# Autodesk Inventor assembly: 000 Ensamblaje hw_DAA - PCB Power
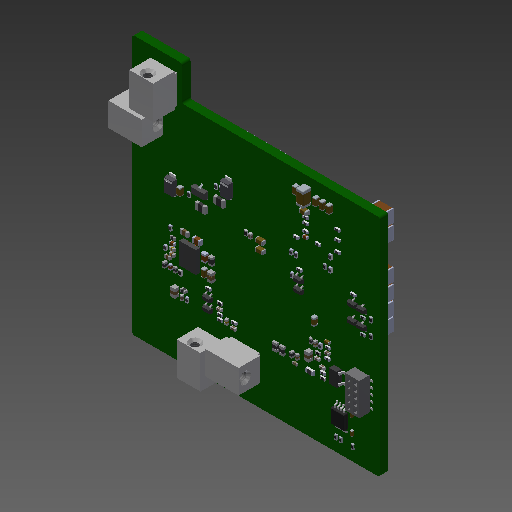
[picture p0: Inventor's stored thumbnail of the model, 512x512]
Saved by Autodesk Inventor 2018 (Build 220112000, 112)
## iProperties
Created: 2024-03-13
Part Number: 000 Ensamblaje hw_DAA - PCB Power
Document SubType Name: Assembly
Designer: cda1
Author: cda1
## Documents named in this file (82)
- C:\Users\cda1\Git\DAA\items\hw_DAA\variants\BASIC\3d\000 Ensamblaje hw_DAA - PCB Power.iam
- C:\Users\cda1\Git\DAA\items\hw_DAA\3d\hw_DAA - PCB Power.ipt
- C:\Users\cda1\Git\DAA\items\_accessories\Componentes PCB\Capacitadores\3d_TDK\3d\CGA9N3X7S2A106K230KB\CGA9N3X7S2A106K230KB.iam
- C:\Users\cda1\Git\DAA\items\_accessories\Componentes PCB\Bobinas\3d_COILCRAFT\3d\XAL7030-472MEC\XAL7030-472MEC.iam
- C:\Users\cda1\Git\DAA\items\_accessories\Componentes PCB\PMIC\TPS65930400RWERQ1\TPS65930400RWERQ1.iam
- C:\Users\cda1\Git\DAA\items\_accessories\Componentes PCB\Mosfet\3d_Vishay\3d\SQJ402EP-T1_GE3.ipt
- C:\Users\cda1\Git\DAA\items\_accessories\Componentes PCB\Mosfet\3d_Vishay\3d\SQJ465EP-T1_GE3\SQJ465EP-T1_GE3.ipt
- C:\Users\cda1\Git\DAA\items\_accessories\Componentes PCB\Inductor\3d_Coilcraft\3d\XAL5030-222MEC\XAL5030-222MEC.ipt
- C:\Users\cda1\Git\DAA\items\_accessories\Componentes PCB\Inductor\3d_Coilcraft\3d\XFL4020-152MEC\XFL4020-152MEC.iam
- C:\Users\cda1\Git\DAA\items\_accessories\Componentes PCB\Inductor\3d_Coilcraft\3d\XEL4020-101MEC\XEL4020-101MEC.iam
- C:\Users\cda1\Git\DAA\items\_accessories\Componentes PCB\Inductor\3d_TDK\3d\XAL4020-601MEC\XAL4020-601MEC.ipt
- C:\Users\cda1\Git\DAA\items\_accessories\Componentes PCB\Capacitadores\3d_Murata Electronics\3d\GCM32EC71A476KE02K\GCM32EC71A476KE02K.ipt
- C:\Users\cda1\Git\DAA\items\_accessories\Componentes PCB\Inductor\3d_TDK\3d\TFM322512ALMAR22MTAA\TFM322512ALMAR22MTAA.iam
- C:\Users\cda1\Git\DAA\items\_accessories\Componentes PCB\Inductor\3d_TDK\3d\TFM322512ALMAR47MTAA\TFM322512ALMAR47MTAA.iam
- C:\Users\cda1\Git\DAA\items\_accessories\Componentes PCB\DC-DC\3d_Texas Instruments\3d\TPS54116QRTWTQ1\TPS54116QRTWTQ1.iam
- C:\Users\cda1\Git\DAA\items\_accessories\Componentes PCB\Conversores\Buck converter\3d_Texas_instruments\TPS62873QWRXSRQ1.iam
- C:\Users\cda1\Git\DAA\items\_accessories\Componentes PCB\Analog Switch\3d_Texas_Instruments\TS5A23157TDGSRQ1\TS5A23157TDGSRQ1.iam
- C:\Users\cda1\Git\DAA\items\_accessories\Componentes PCB\Capacitadores\3d_Taiyo Yuden\3d\EMK212BBJ106KGHT.ipt
- C:\Users\cda1\Git\DAA\items\_accessories\Componentes PCB\Capacitadores\3d_Murata Electronics\3d\GRT32ER60J107ME13L.ipt
- C:\Users\cda1\Git\DAA\items\_accessories\Componentes PCB\Condensadores\3d_TDK\3d\CGA6P3X7S1H685M250AB\CGA6P3X7S1H685M250AB.iam
- C:\Users\cda1\Git\DAA\items\_accessories\Componentes PCB\Capacitadores\3d_Murata Electronics\3d\GRM31CC72A475ME11L.ipt
- C:\Users\cda1\Git\DAA\items\_accessories\Componentes PCB\Reguladores\3d_Texas Instruments\3d\TPS57112CQRTERQ1\TPS57112CQRTERQ1.iam
- C:\Users\cda1\Git\DAA\items\_accessories\Componentes PCB\Reguladores\3d_Texas Instruments\3d\TPS74525PQWDRBRQ1\TPS74525PQWDRBRQ1.iam
- C:\Users\cda1\Git\DAA\items\_accessories\Componentes PCB\Cristales\3d_ECS\3d\ECS-.327-12.5-34QCS-TR\ECS-.327-12.5-34QCS-TR.ipt
- C:\Users\cda1\Git\DAA\items\_accessories\Componentes PCB\Diodos\3d_Semtech\3d\RCLAMP3324PQTCT\RCLAMP3324PQTCT.ipt
- C:\Users\cda1\Git\DAA\items\_accessories\Componentes PCB\Resistencias\3d_Vishay\3d\CRCW12061R00FKEAHP\CRCW12061R00FKEAHP.iam
- C:\Users\cda1\Git\DAA\items\_accessories\Componentes PCB\Resistencias\3d_Vishay\3d\CMB02070X1000GB200\CMB02070X1000GB200.ipt
- C:\Users\cda1\Git\DAA\items\_accessories\Componentes PCB\Capacitadores\3d_TDK\3d\CGA3E1X7S1C225K080AC\CGA3E1X7S1C225K080AC.iam
- C:\Users\cda1\Git\DAA\items\_accessories\Componentes PCB\Capacitadores\3d_Murata Electronics\3d\GCM1555C1H120JA16J\GCM1555C1H120JA16J.iam
- C:\Users\cda1\Git\DAA\items\_accessories\Componentes PCB\Capacitadores\3d_TDK\3d\CGA2B3X7R1H104K050BD.ipt
- C:\Users\cda1\Git\DAA\items\_accessories\Componentes PCB\Capacitadores\3d_Murata Electronics\3d\GRT188C81A106ME13D.ipt
- C:\Users\cda1\Git\DAA\items\_accessories\Componentes PCB\Capacitadores\3d_Taiyo Yuden\3d\HMJ107BB7104KAHT.ipt
- C:\Users\cda1\Git\DAA\items\_accessories\Componentes PCB\Capacitadores\3d_Genérico\3d\CAPC-0402-T0.55-BN.ipt
- C:\Users\cda1\Git\DAA\items\_accessories\Componentes PCB\Capacitadores\3d_Murata Electronics\3d\GCM1555C1H121JA16D\GCM1555C1H121JA16D.ipt
- C:\Users\cda1\Git\DAA\items\_accessories\Componentes PCB\Resistencias\3d_Panasonic\3d\ERJ-2GE0R00X.ipt
- C:\Users\cda1\Git\DAA\items\_accessories\Componentes PCB\Resistencias\3d_Panasonic\3d\ERJ-2RKF2002X\ERJ-2RKF2002X.iam
- C:\Users\cda1\Git\DAA\items\_accessories\Componentes PCB\Resistencias\3d_Vishay\3d\CRCW04028K66FKTD\CRCW04028K66FKTD.ipt
- C:\Users\cda1\Git\DAA\items\_accessories\Componentes PCB\Resistencias\3d_Panasonic\3d\ERJ-2RKF1543X\ERJ-2RKF1543X.iam
- C:\Users\cda1\Git\DAA\items\_accessories\Componentes PCB\Resistencias\3d_Genérico\RESC-0402.ipt
- C:\Users\cda1\Git\DAA\items\_accessories\Componentes PCB\Resistencias\3d_Panasonic\3d\ERJ-2RKF1002X.ipt
- C:\Users\cda1\Git\DAA\items\_accessories\Componentes PCB\Conectores\3d_Samtec\3d\CLP-105-02-F-D-BE\CLP-105-02-F-D-BE.iam
- C:\Users\cda1\Git\DAA\items\_accessories\Componentes PCB\Capacitadores\3d_Murata Electronics\3d\GRT31CC81C226KE01L.ipt
- C:\Users\cda1\Git\DAA\items\_accessories\Componentes PCB\Elementos mecanicos soldables\3d_Wurth Electronics\3d\SMD\WP-SMRA Redcube (M2) 7466302.ipt
- C:\Users\cda1\Git\DAA\items\_accessories\Componentes PCB\Elementos mecanicos soldables\3d_Wurth Electronics\3d\SMD\WP-SMRA Redcube (M2) 746630200.ipt
- C:\Users\cda1\Git\DAA\items\_accessories\Componentes PCB\DC-DC\3d_Texas Instruments\3d\LM5146QRGYRQ1\LM5146QRGYRQ1.iam
- C:\Users\cda1\Git\DAA\items\_accessories\Componentes PCB\I2C\3d_Texas_Instruments\TCA9517DGKRQ1\TCA9517DGKRQ1.iam
- C:\Users\cda1\Git\DAA\items\_accessories\Componentes PCB\Diodos\3d_Diodes Incorporated\3d\DMN2710UTQ-7\DMN2710UTQ-7.ipt
- C:\Users\cda1\Git\DAA\items\_accessories\Componentes PCB\Mosfet\3d_Infineon\3d\BSS123NH6327XTSA1\BSS123NH6327XTSA1.iam
- C:\Users\cda1\Git\DAA\items\_accessories\Componentes PCB\Diodos\3d_Vishay\3d\BZD27C10P-HE3-08.ipt
- C:\Users\cda1\Git\DAA\items\_accessories\Componentes PCB\Capacitadores\3d_Kemet\3d\C0603C105K4RACAUTO.ipt
- C:\Users\cda1\Git\DAA\items\_accessories\Componentes PCB\Capacitadores\3d_TDK\3d\CGA2B1X7S1C474K050BC.ipt
- C:\Users\cda1\Git\DAA\items\_accessories\Componentes PCB\Capacitadores\3d_Murata Electronics\3d\GCM155R71C563KA55J\GCM155R71C563KA55J.ipt
- C:\Users\cda1\Git\DAA\items\_accessories\Componentes PCB\Capacitadores\3d_Kemet\3d\C0402C822K4RACAUTO\C0402C822K4RACAUTO.ipt
- C:\Users\cda1\Git\DAA\items\_accessories\Componentes PCB\Capacitadores\3d_Murata Electronics\3d\GCG155R71H821KA01D\GCG155R71H821KA01D.ipt
- C:\Users\cda1\Git\DAA\items\_accessories\Componentes PCB\Capacitadores\3d_Murata Electronics\3d\GCM155R71H391KA37D\GCM155R71H391KA37D.ipt
- C:\Users\cda1\Git\DAA\items\_accessories\Componentes PCB\Capacitadores\3d_Kyocera\3d\06031A6R8J4T4A\06031A6R8J4T4A.ipt
- C:\Users\cda1\Git\DAA\items\_accessories\Componentes PCB\Capacitadores\3d_Kemet\3d\C0603X272J5GAC7867\C0603X272J5GAC7867.ipt
- C:\Users\cda1\Git\DAA\items\_accessories\Componentes PCB\Capacitadores\3d_TDK\3d\CGA2B1X7R1V224K050BC\CGA2B1X7R1V224K050BC.iam
- C:\Users\cda1\Git\DAA\items\_accessories\Componentes PCB\Capacitadores\3d_Murata Electronics\3d\GRT155R71H331KE01D\GRT155R71H331KE01D.ipt
- C:\Users\cda1\Git\DAA\items\_accessories\Componentes PCB\Capacitadores\3d_AVX\3d\04025A220C4T2A.ipt
- C:\Users\cda1\Git\DAA\items\_accessories\Componentes PCB\Capacitadores\3d_Murata Electronics\3d\GCM155R71H332KA37J\GCM155R71H332KA37J.ipt
- C:\Users\cda1\Git\DAA\items\_accessories\Componentes PCB\Capacitadores\3d_Murata Electronics\3d\GCQ1555C1H100FB01D\GCQ1555C1H100FB01D.ipt
- C:\Users\cda1\Git\DAA\items\_accessories\Componentes PCB\Condensadores\3d-Murata\3d\GCM155R72A472MA37D\GCM155R72A472MA37D.ipt
- C:\Users\cda1\Git\DAA\items\_accessories\Componentes PCB\Resistencias\3d_Yageo\3d\AC0805FR-0749K9L\AC0805FR-0749K9L.ipt
- C:\Users\cda1\Git\DAA\items\_accessories\Componentes PCB\Resistencias\3d_Panasonic\3d\ERJ-2RKF1003X.ipt
- C:\Users\cda1\Git\DAA\items\_accessories\Componentes PCB\Resistencias\3d_Panasonic\3d\ERJ-U02F4701X\ERJ-U02F4701X.iam
- C:\Users\cda1\Git\DAA\items\_accessories\Componentes PCB\Resistencias\3d_Vishay\3d\CRCW040233K0FKED\CRCW040233K0FKED.ipt
- C:\Users\cda1\Git\DAA\items\_accessories\Componentes PCB\Diodos\3d_Vishay\3d\GSOT05C-HE3-08.ipt
- C:\Users\cda1\Git\DAA\items\_accessories\Componentes PCB\Resistencias\3d_Vishay\3d\CRCW060315K0FKEA.ipt
- C:\Users\cda1\Git\DAA\items\_accessories\Componentes PCB\Resistencias\3d_Panasonic\3d\ERJ-2RKF9090X\ERJ-2RKF9090X.ipt
- C:\Users\cda1\Git\DAA\items\_accessories\Componentes PCB\Resistencias\3d_Vishay\3d\CRCW06036K19FKEA\CRCW06036K19FKEA.ipt
- C:\Users\cda1\Git\DAA\items\_accessories\Componentes PCB\Resistencias\3d_TE Connectivity\3d\CRGP0402F47K.ipt
- C:\Users\cda1\Git\DAA\items\_accessories\Componentes PCB\Resistencias\3d_Vishay\3d\CRCW0402110KFKTD\CRCW0402110KFKTD.ipt
- C:\Users\cda1\Git\DAA\items\_accessories\Componentes PCB\Resistencias\3d_Yageo\3d\AC0402FR-0797K6L.ipt
- C:\Users\cda1\Git\DAA\items\_accessories\Componentes PCB\Resistencias\3d_Vishay\3d\CRCW040278K7FKTD\CRCW040278K7FKTD.ipt
- C:\Users\cda1\Git\DAA\items\_accessories\Componentes PCB\Resistencias\3d_Vishay\3d\CRCW04023K40FKED\CRCW04023K40FKED.ipt
- C:\Users\cda1\Git\DAA\items\_accessories\Componentes PCB\Resistencias\3d_Vishay\3d\CRCW0402133RFKED\CRCW0402133RFKED.ipt
- C:\Users\cda1\Git\DAA\items\_accessories\Componentes PCB\Resistencias\3d_KOA\3d\RK73H1ETTP1802F\RK73H1ETTP1802F.ipt
- C:\Users\cda1\Git\DAA\items\_accessories\Componentes PCB\Resistencias\3d_Panasonic\3d\ERJ-2RKF1501X.ipt
- C:\Users\cda1\Git\DAA\items\_accessories\Componentes PCB\Resistencias\3d_Vishay\3d\CRCW040239K2FKED\CRCW040239K2FKED.ipt
- C:\Users\cda1\Git\DAA\items\_accessories\Componentes PCB\Resistencias\3d_Vishay\3d\CRCW06032R10FKEA\CRCW06032R10FKEA.ipt
- C:\Users\cda1\Git\DAA\items\_accessories\Componentes PCB\Resistencias\3d_Vishay\3d\CRCW0603931RFKEA\CRCW0603931RFKEA.ipt
## Components (216 placed, 81 different names)
1. hw_DAA - PCB Power:1 — Coincidencia:51, Coincidencia:52, Coincidencia:53, Coincidencia:54, Coincidencia:55, Coincidencia:56, Coincidencia:57, Coincidencia:58, Coincidencia:59, Coincidencia:60, Coincidencia:61, Coincidencia:62, Coincidencia:63, Coincidencia:64, Coincidencia:65, Coincidencia:66, Coincidencia:67, Coincidencia:68, Coincidencia:69, Coincidencia:70, Coincidencia:71, Coincidencia:72, Coincidencia:73, Coincidencia:74, Coincidencia:75, Coincidencia:76, Coincidencia:77, Coincidencia:78, Coincidencia:79, Coincidencia:80, Coincidencia:81, Coincidencia:82, Coincidencia:83, Coincidencia:84, Coincidencia:85, Coincidencia:86, Coincidencia:87, Coincidencia:88, Coincidencia:89, Ángulo:1, Ángulo:2, Coincidencia:90, Ángulo:3, Coincidencia:91, Coincidencia:92, Coincidencia:93, Coincidencia:94, Coincidencia:95, Coincidencia:96, Coincidencia:97, Ángulo:4, Ángulo:5, Coincidencia:98, Ángulo:6, Coincidencia:99, Ángulo:7, Coincidencia:100, Coincidencia:101, Ángulo:8, Ángulo:9, Coincidencia:102, Coincidencia:103, Coincidencia:104, Coincidencia:105, Coincidencia:106, Coincidencia:107, Ángulo:10, Ángulo:11, Coincidencia:108, Coincidencia:109, Ángulo:12, Ángulo:13, Tangente:1, Ángulo:14, Coincidencia:110, Ángulo:15, Coincidencia:111, Coincidencia:112, Coincidencia:113, Coincidencia:114, Coincidencia:115, Coincidencia:116, Ángulo:16, Coincidencia:117, Coincidencia:118, Coincidencia:119, Coincidencia:120, Coincidencia:121, Ángulo:17, Coincidencia:122, Coincidencia:123, Coincidencia:124, Ángulo:18, Coincidencia:125, Coincidencia:126, Ángulo:19, Coincidencia:127, Ángulo:20, Coincidencia:128, Coincidencia:129, Coincidencia:130, Coincidencia:131, Coincidencia:132, Coincidencia:133, Coincidencia:134, Coincidencia:135, Coincidencia:136, Coincidencia:137, Coincidencia:138, Coincidencia:139, Ángulo:21, Coincidencia:140, Ángulo:22, Coincidencia:141, Ángulo:23, Coincidencia:149, Ángulo:24, Coincidencia:151, Ángulo:25, Coincidencia:153, Ángulo:26, Coincidencia:154, Coincidencia:155, Coincidencia:156, Coincidencia:157, Coincidencia:158, Coincidencia:159, Coincidencia:160, Coincidencia:161, Coincidencia:162, Ángulo:27, Ángulo:28, Coincidencia:163, Coincidencia:164, Coincidencia:165, Ángulo:29, Coincidencia:166, Ángulo:30, Coincidencia:167, Coincidencia:168, Ángulo:31, Coincidencia:169, Coincidencia:170, Coincidencia:171, Coincidencia:172, Coincidencia:173, Coincidencia:174, Ángulo:32, Coincidencia:175, Coincidencia:176, Coincidencia:177, Ángulo:33, Coincidencia:178, Coincidencia:179, Coincidencia:180, Coincidencia:181, Ángulo:34, Coincidencia:182, Ángulo:35, Coincidencia:183, Ángulo:36, Coincidencia:184, Ángulo:37, Coincidencia:185, Ángulo:38, Coincidencia:186, Ángulo:39, Coincidencia:187, Coincidencia:188, Coincidencia:189, Ángulo:40, Coincidencia:190, Coincidencia:191, Coincidencia:192, Coincidencia:193, Ángulo:41, Ángulo:42, Coincidencia:195, Ángulo:43, Coincidencia:196, Ángulo:44, Coincidencia:197, Coincidencia:198, Coincidencia:200, Coincidencia:201, Coincidencia:202, Coincidencia:203, Ángulo:45, Coincidencia:204, Ángulo:46, Coincidencia:205, Coincidencia:206, Coincidencia:207, Coincidencia:208, Coincidencia:209, Ángulo:47, Coincidencia:210, Coincidencia:211, Coincidencia:212, Coincidencia:213, Coincidencia:214, Coincidencia:215, Coincidencia:216, Ángulo:48, Ángulo:49, Coincidencia:217, Coincidencia:218, Ángulo:50, Coincidencia:219, Coincidencia:220, Coincidencia:221, Coincidencia:222, Coincidencia:223, Ángulo:51, Ángulo:52, Coincidencia:224, Ángulo:53, Coincidencia:225, Ángulo:54, Coincidencia:226, Coincidencia:227, Coincidencia:228, Coincidencia:229, Coincidencia:230, Coincidencia:231, Coincidencia:232, Coincidencia:233, Coincidencia:234, Coincidencia:235, Coincidencia:236, Coincidencia:237, Coincidencia:238, Coincidencia:239, Coincidencia:240, Coincidencia:241, Coincidencia:242, Coincidencia:243, Coincidencia:244, Coincidencia:245, Coincidencia:250, Coincidencia:251, Coincidencia:252, Coincidencia:253, Coincidencia:254, Coincidencia:255, Coincidencia:256, Coincidencia:257, Coincidencia:258, Coincidencia:259, Coincidencia:260, Ángulo:55, Coincidencia:261, Coincidencia:262, Ángulo:56, Coincidencia:263, Coincidencia:264, Ángulo:57, Nivelación:1, Nivelación:4, Ángulo:58, Ángulo:59, Ángulo:60, Ángulo:61, Ángulo:62, Ángulo:63, Coincidencia:266, Coincidencia:267, Coincidencia:268, Coincidencia:269, Coincidencia:270, Coincidencia:271, Coincidencia:272, Ángulo:64, Ángulo:65, Coincidencia:273, Coincidencia:274, Coincidencia:275, Coincidencia:276, Ángulo:66, Coincidencia:277, Coincidencia:278, Ángulo:67, Coincidencia:279, Coincidencia:281, Coincidencia:283, Coincidencia:284, Ángulo:68, Coincidencia:285, Coincidencia:286, Coincidencia:287, Ángulo:69, Ángulo:70
2. CGA9N3X7S2A106K230KB:1 [sub-assembly] — Coincidencia:51
3. CGA9N3X7S2A106K230KB:2 [sub-assembly] — Coincidencia:53
4. CGA9N3X7S2A106K230KB:3 [sub-assembly] — Coincidencia:52
5. XAL7030-472MEC:1 [sub-assembly] — Coincidencia:54
6. XAL7030-472MEC:2 [sub-assembly] — Coincidencia:55
7. TPS65930400RWERQ1:1 [sub-assembly] — Coincidencia:56
8. SQJ402EP-T1_GE3:1 — Coincidencia:57, Coincidencia:60
9. SQJ402EP-T1_GE3:2 — Coincidencia:58, Coincidencia:59
10. SQJ465EP-T1_GE3:1 — Coincidencia:61
11. XAL5030-222MEC:1 — Coincidencia:62
12. XFL4020-152MEC:1 [sub-assembly] — Coincidencia:63
13. XEL4020-101MEC:1 [sub-assembly] — Coincidencia:64
14. XAL4020-601MEC:1 — Coincidencia:65
15. GCM32EC71A476KE02K:1 — Coincidencia:69
16. GCM32EC71A476KE02K:2 — Coincidencia:68
17. GCM32EC71A476KE02K:3 — Coincidencia:67
18. GCM32EC71A476KE02K:4 — Coincidencia:66
19. GCM32EC71A476KE02K:5 — Coincidencia:71, Ángulo:58
20. GCM32EC71A476KE02K:6 — Coincidencia:70, Ángulo:59
21. GCM32EC71A476KE02K:7 — Coincidencia:72, Ángulo:60
22. TFM322512ALMAR22MTAA:1 [sub-assembly] — Coincidencia:74
23. TFM322512ALMAR22MTAA:2 [sub-assembly] — Coincidencia:73
24. TFM322512ALMAR47MTAA:1 [sub-assembly] — Coincidencia:75
25. TFM322512ALMAR47MTAA:2 [sub-assembly] — Coincidencia:76
26. TFM322512ALMAR22MTAA:3 [sub-assembly] — Coincidencia:77
27. TPS54116QRTWTQ1:1 [sub-assembly] — Coincidencia:78
28. TPS62873QWRXSRQ1:1 [sub-assembly] — Coincidencia:79
29. TS5A23157TDGSRQ1:1 [sub-assembly] — Coincidencia:80, Coincidencia:81
30. EMK212BBJ106KGHT:1 — Coincidencia:84
31. EMK212BBJ106KGHT:2 — Coincidencia:85
32. EMK212BBJ106KGHT:3 — Coincidencia:83
33. EMK212BBJ106KGHT:4 — Coincidencia:82
34. GCM32EC71A476KE02K:8 — Coincidencia:86
35. GCM32EC71A476KE02K:9 — Coincidencia:87
36. GRT32ER60J107ME13L:1 — Coincidencia:89, Ángulo:1
37. GCM32EC71A476KE02K:10 — Coincidencia:88, Ángulo:2
38. GRT32ER60J107ME13L:2 — Coincidencia:90, Ángulo:3
39. CGA6P3X7S1H685M250AB:1 [sub-assembly] — Coincidencia:91
40. CGA6P3X7S1H685M250AB:2 [sub-assembly] — Coincidencia:92
41. GCM32EC71A476KE02K:11 — Coincidencia:93
42. GCM32EC71A476KE02K:12 — Coincidencia:94
43. GCM32EC71A476KE02K:13 — Coincidencia:95
44. GRM31CC72A475ME11L:1 — Coincidencia:96, Ángulo:5
45. GRM31CC72A475ME11L:2 — Coincidencia:97, Ángulo:4
46. GRT32ER60J107ME13L:3 — Coincidencia:98, Ángulo:6
47. GCM32EC71A476KE02K:14 — Coincidencia:99, Ángulo:7
48. GRM31CC72A475ME11L:3 — Coincidencia:101, Ángulo:8
49. GRM31CC72A475ME11L:4 — Coincidencia:100, Ángulo:9
50. TPS57112CQRTERQ1:1 [sub-assembly] — Coincidencia:102
51. TPS57112CQRTERQ1:2 [sub-assembly] — Coincidencia:103
52. TPS74525PQWDRBRQ1:1 [sub-assembly] — Coincidencia:104
53. ECS-.327-12.5-34QCS-TR:1 — Coincidencia:105
54. RCLAMP3324PQTCT:1 — Coincidencia:107, Ángulo:10
55. RCLAMP3324PQTCT:2 — Coincidencia:106, Ángulo:11
56. CRCW12061R00FKEAHP:1 [sub-assembly] — Coincidencia:108, Ángulo:13
57. CRCW12061R00FKEAHP:2 [sub-assembly] — Coincidencia:109, Ángulo:12
58. CMB02070X1000GB200:1 — Tangente:1, Ángulo:14
59. CGA3E1X7S1C225K080AC:1 [sub-assembly] — Coincidencia:110, Ángulo:15
60. CGA3E1X7S1C225K080AC:2 [sub-assembly] — Coincidencia:111
61. CGA3E1X7S1C225K080AC:3 [sub-assembly] — Coincidencia:112
62. CGA3E1X7S1C225K080AC:4 [sub-assembly] — Coincidencia:113
63. CGA3E1X7S1C225K080AC:5 [sub-assembly] — Coincidencia:114
64. CGA3E1X7S1C225K080AC:6 [sub-assembly] — Coincidencia:115
65. EMK212BBJ106KGHT:5 — Coincidencia:116, Ángulo:16
66. GCM1555C1H120JA16J:1 [sub-assembly] — Coincidencia:118
67. GCM1555C1H120JA16J:2 [sub-assembly] — Coincidencia:117
68. CGA2B3X7R1H104K050BD:1 — Coincidencia:119
69. GRT188C81A106ME13D:1 — Coincidencia:120
70. GRT188C81A106ME13D:2 — Coincidencia:121, Ángulo:17
71. GRT188C81A106ME13D:3 — Coincidencia:122
72. GRT188C81A106ME13D:4 — Coincidencia:123
73. HMJ107BB7104KAHT:1 — Coincidencia:124, Ángulo:18
74. CAPC-0402-T0.55-BN:1 — Coincidencia:125
75. CGA2B3X7R1H104K050BD:2 — Coincidencia:126, Ángulo:19
76. HMJ107BB7104KAHT:2 — Coincidencia:127, Ángulo:20
77. HMJ107BB7104KAHT:3 — Coincidencia:128
78. GCM1555C1H121JA16D:1 — Coincidencia:129
79. CAPC-0402-T0.55-BN:2 — Coincidencia:130
80. CGA2B3X7R1H104K050BD:3 — Coincidencia:131
81. HMJ107BB7104KAHT:4 — Coincidencia:132
82. ERJ-2GE0R00X:1 — Coincidencia:133
83. ERJ-2RKF2002X:1 [sub-assembly] — Coincidencia:134
84. CRCW04028K66FKTD:1 — Coincidencia:135
85. ERJ-2RKF1543X:1 [sub-assembly] — Coincidencia:136
86. RESC-0402:1 — Coincidencia:137
87. RESC-0402:2 — Coincidencia:138
88. ERJ-2RKF1002X:1 — Coincidencia:139, Ángulo:21
89. ERJ-2RKF1002X:2 — Coincidencia:140, Ángulo:22
90. CLP-105-02-F-D-BE:1 [sub-assembly] — Coincidencia:141, Ángulo:23
91. GCM32EC71A476KE02K:15 — Ángulo:63, Coincidencia:268
92. GCM32EC71A476KE02K:16 — Coincidencia:271, Ángulo:64
93. GCM32EC71A476KE02K:17 — Coincidencia:270
94. GCM32EC71A476KE02K:18 — Coincidencia:269
95. GCM32EC71A476KE02K:19 — Ángulo:61, Coincidencia:267
96. GCM32EC71A476KE02K:20 — Ángulo:62, Coincidencia:266
97. GCM32EC71A476KE02K:21 — Coincidencia:272, Ángulo:65
98. GRT31CC81C226KE01L:1 — Coincidencia:149, Ángulo:24
99. WP-SMRA Redcube (M2) 746630200:3
100. WP-SMRA Redcube (M2) 7466302:2 — Coincidencia:151, Ángulo:25, Nivelación:1, Coincidencia:281
101. WP-SMRA Redcube (M2) 746630200:2
102. WP-SMRA Redcube (M2) 746630200:1 — Coincidencia:153, Ángulo:26, Nivelación:4, Coincidencia:283
103. LM5146QRGYRQ1:1 [sub-assembly] — Coincidencia:154
104. TCA9517DGKRQ1:1 [sub-assembly] — Coincidencia:155, Coincidencia:156
105. DMN2710UTQ-7:1 — Coincidencia:157
106. DMN2710UTQ-7:2 — Coincidencia:158
107. DMN2710UTQ-7:3 — Coincidencia:161, Ángulo:27
108. DMN2710UTQ-7:4 — Coincidencia:159
109. DMN2710UTQ-7:5 — Coincidencia:162, Ángulo:28
110. DMN2710UTQ-7:6 — Coincidencia:160
111. DMN2710UTQ-7:7 — Coincidencia:163
112. DMN2710UTQ-7:8 — Coincidencia:164
113. BSS123NH6327XTSA1:1 [sub-assembly] — Coincidencia:165, Ángulo:29
114. BZD27C10P-HE3-08:1 — Coincidencia:166, Ángulo:30
115. BZD27C10P-HE3-08:2 — Coincidencia:167
116. CGA3E1X7S1C225K080AC:7 [sub-assembly] — Coincidencia:168, Ángulo:31
117. CGA3E1X7S1C225K080AC:8 [sub-assembly] — Coincidencia:169
118. CGA3E1X7S1C225K080AC:9 [sub-assembly] — Coincidencia:170
119. CGA3E1X7S1C225K080AC:10 [sub-assembly] — Coincidencia:171
120. C0603C105K4RACAUTO:1 — Coincidencia:172
121. CGA2B1X7S1C474K050BC:1 — Coincidencia:173
122. CGA3E1X7S1C225K080AC:11 [sub-assembly] — Coincidencia:174, Ángulo:32
123. CGA3E1X7S1C225K080AC:12 [sub-assembly] — Coincidencia:175
124. CGA3E1X7S1C225K080AC:13 [sub-assembly] — Coincidencia:176
125. CAPC-0402-T0.55-BN:3 — Coincidencia:177, Ángulo:33
126. GCM155R71C563KA55J:1 — Coincidencia:178
127. C0402C822K4RACAUTO:1 — Coincidencia:179
128. GCG155R71H821KA01D:1 — Coincidencia:180
129. GCM155R71H391KA37D:1 — Coincidencia:181, Ángulo:34
130. HMJ107BB7104KAHT:5 — Coincidencia:182, Ángulo:35
131. 06031A6R8J4T4A:1 — Coincidencia:183, Ángulo:36
132. CGA3E1X7S1C225K080AC:14 [sub-assembly] — Coincidencia:184, Ángulo:37
133. C0603X272J5GAC7867:1 — Coincidencia:185, Ángulo:38
134. CAPC-0402-T0.55-BN:4 — Coincidencia:186, Ángulo:39
135. HMJ107BB7104KAHT:6 — Coincidencia:187
136. CAPC-0402-T0.55-BN:5 — Coincidencia:188
137. C0402C822K4RACAUTO:2 — Coincidencia:189, Ángulo:40
138. CGA2B1X7R1V224K050BC:1 [sub-assembly] — Coincidencia:190
139. GRT155R71H331KE01D:1 — Coincidencia:191
140. 04025A220C4T2A:1 — Coincidencia:192
141. GCM155R71H332KA37J:1 — Coincidencia:193, Ángulo:41
142. GCM155R71H332KA37J:2 — Ángulo:42, Coincidencia:286
143. C0603X272J5GAC7867:2 — Coincidencia:195, Ángulo:43
144. GCQ1555C1H100FB01D:1 — Coincidencia:196, Ángulo:44
145. GCM155R72A472MA37D:1 — Coincidencia:197
146. 04025A220C4T2A:2 — Coincidencia:198
147. CAPC-0402-T0.55-BN:6 — Coincidencia:278, Ángulo:67
148. CAPC-0402-T0.55-BN:7 — Coincidencia:200
149. AC0805FR-0749K9L:1 — Coincidencia:201
150. AC0805FR-0749K9L:2 — Coincidencia:202
151. RESC-0402:3 — Coincidencia:203, Ángulo:45
152. ERJ-2RKF1003X:1 — Coincidencia:204, Ángulo:46
153. ERJ-2RKF1003X:2 — Coincidencia:205
154. ERJ-2GE0R00X:2 — Coincidencia:206
155. ERJ-2GE0R00X:3 — Coincidencia:207
156. ERJ-2RKF1002X:3 — Coincidencia:208
157. ERJ-2RKF1002X:4 — Coincidencia:209, Ángulo:47
158. ERJ-2GE0R00X:4 — Coincidencia:210
159. ERJ-2RKF1002X:5 — Coincidencia:211
160. ERJ-2GE0R00X:5 — Coincidencia:212
161. ERJ-2GE0R00X:6 — Coincidencia:213
162. ERJ-2GE0R00X:7 — Coincidencia:214
163. ERJ-2GE0R00X:8 — Coincidencia:215, Ángulo:49
164. ERJ-2GE0R00X:9 — Coincidencia:216, Ángulo:48
165. ERJ-2RKF1002X:6 — Coincidencia:217
166. ERJ-2RKF1002X:7 — Coincidencia:218, Ángulo:50
167. ERJ-2RKF1002X:8 — Coincidencia:219
168. ERJ-U02F4701X:1 [sub-assembly] — Coincidencia:220
169. ERJ-U02F4701X:2 [sub-assembly] — Coincidencia:222, Ángulo:51
170. ERJ-U02F4701X:3 [sub-assembly] — Coincidencia:221
171. ERJ-U02F4701X:4 [sub-assembly] — Coincidencia:223, Ángulo:52
172. C0603C105K4RACAUTO:2 — Coincidencia:224, Ángulo:53
173. CRCW040233K0FKED:1 — Coincidencia:225, Ángulo:54
174. GSOT05C-HE3-08:1 — Coincidencia:230, Coincidencia:231
175. ERJ-2RKF1002X:9 — Coincidencia:227
176. CRCW04028K66FKTD:2 — Coincidencia:228
177. ERJ-2RKF1002X:10 — Coincidencia:229
178. ERJ-2RKF1003X:3 — Coincidencia:226
179. CGA2B3X7R1H104K050BD:4 — Coincidencia:232
180. CGA2B3X7R1H104K050BD:5 — Coincidencia:233
181. ERJ-U02F4701X:5 [sub-assembly] — Coincidencia:238
182. ERJ-U02F4701X:6 [sub-assembly] — Coincidencia:237
183. ERJ-U02F4701X:7 [sub-assembly] — Coincidencia:239
184. ERJ-U02F4701X:8 [sub-assembly] — Coincidencia:240
185. ERJ-2RKF1002X:11 — Coincidencia:236
186. CRCW060315K0FKEA:1 — Coincidencia:242
187. ERJ-2RKF1002X:12 — Coincidencia:234
188. RESC-0402:4 — Coincidencia:235
189. ERJ-2RKF9090X:1 — Coincidencia:241
190. CRCW06036K19FKEA:1 — Coincidencia:243
191. CRCW06036K19FKEA:2 — Coincidencia:244
192. ERJ-2RKF1002X:13 — Coincidencia:245
193. ERJ-2RKF1003X:4 — Coincidencia:276, Ángulo:66
194. ERJ-2RKF1003X:5 — Coincidencia:251
195. RESC-0402:5 — Coincidencia:250
196. ERJ-2RKF1003X:6 — Coincidencia:252
197. CRGP0402F47K:1 — Coincidencia:277
198. CRCW0402110KFKTD:1 — Coincidencia:287, Ángulo:69
199. ERJ-2RKF1003X:7 — Coincidencia:285, Ángulo:70
200. AC0402FR-0797K6L:1 — Coincidencia:253
201. CRCW040278K7FKTD:1 — Coincidencia:254
202. CRCW04023K40FKED:1 — Coincidencia:256
203. CRCW0402133RFKED:1 — Coincidencia:257
204. RESC-0402:6 — Coincidencia:255
205. RK73H1ETTP1802F:1 — Coincidencia:258
206. ERJ-2RKF1002X:14 — Coincidencia:259
207. ERJ-2RKF1501X:1 — Coincidencia:260, Ángulo:55
208. CRCW040239K2FKED:1 — Coincidencia:261
209. ERJ-2RKF1003X:8 — Coincidencia:262, Ángulo:56
210. CRCW06032R10FKEA:1 — Coincidencia:263
211. CRCW0603931RFKEA:1 — Coincidencia:264, Ángulo:57
212. GRT32ER60J107ME13L:4 — Coincidencia:273
213. CGA2B3X7R1H104K050BD:6 — Coincidencia:274
214. C0603X272J5GAC7867:3 — Coincidencia:275
215. CGA2B3X7R1H104K050BD:7 — Coincidencia:279
216. ERJ-2RKF1003X:9 — Coincidencia:284, Ángulo:68
## Relationships (298: Mate 223, Angle 70, Flush 4, Tangent 1)
- Coincidencia:51 [Mate]: hw_DAA - PCB Power:1 ↔ CGA9N3X7S2A106K230KB:1
- Coincidencia:52 [Mate]: hw_DAA - PCB Power:1 ↔ CGA9N3X7S2A106K230KB:3
- Coincidencia:53 [Mate]: hw_DAA - PCB Power:1 ↔ CGA9N3X7S2A106K230KB:2
- Coincidencia:54 [Mate]: hw_DAA - PCB Power:1 ↔ XAL7030-472MEC:1
- Coincidencia:55 [Mate]: hw_DAA - PCB Power:1 ↔ XAL7030-472MEC:2
- Coincidencia:56 [Mate]: hw_DAA - PCB Power:1 ↔ TPS65930400RWERQ1:1
- Coincidencia:57 [Mate]: hw_DAA - PCB Power:1 ↔ SQJ402EP-T1_GE3:1
- Coincidencia:58 [Mate]: hw_DAA - PCB Power:1 ↔ SQJ402EP-T1_GE3:2
- Coincidencia:59 [Mate]: hw_DAA - PCB Power:1 ↔ SQJ402EP-T1_GE3:2
- Coincidencia:60 [Mate]: hw_DAA - PCB Power:1 ↔ SQJ402EP-T1_GE3:1
- Coincidencia:61 [Mate]: hw_DAA - PCB Power:1 ↔ SQJ465EP-T1_GE3:1
- Coincidencia:62 [Mate]: hw_DAA - PCB Power:1 ↔ XAL5030-222MEC:1
- Coincidencia:63 [Mate]: hw_DAA - PCB Power:1 ↔ XFL4020-152MEC:1
- Coincidencia:64 [Mate]: hw_DAA - PCB Power:1 ↔ XEL4020-101MEC:1
- Coincidencia:65 [Mate]: hw_DAA - PCB Power:1 ↔ XAL4020-601MEC:1
- Coincidencia:66 [Mate]: hw_DAA - PCB Power:1 ↔ GCM32EC71A476KE02K:4
- Coincidencia:67 [Mate]: hw_DAA - PCB Power:1 ↔ GCM32EC71A476KE02K:3
- Coincidencia:68 [Mate]: hw_DAA - PCB Power:1 ↔ GCM32EC71A476KE02K:2
- Coincidencia:69 [Mate]: hw_DAA - PCB Power:1 ↔ GCM32EC71A476KE02K:1
- Coincidencia:70 [Mate]: hw_DAA - PCB Power:1 ↔ GCM32EC71A476KE02K:6
- Coincidencia:71 [Mate]: hw_DAA - PCB Power:1 ↔ GCM32EC71A476KE02K:5
- Coincidencia:72 [Mate]: hw_DAA - PCB Power:1 ↔ GCM32EC71A476KE02K:7
- Coincidencia:73 [Mate]: hw_DAA - PCB Power:1 ↔ TFM322512ALMAR22MTAA:2
- Coincidencia:74 [Mate]: hw_DAA - PCB Power:1 ↔ TFM322512ALMAR22MTAA:1
- Coincidencia:75 [Mate]: hw_DAA - PCB Power:1 ↔ TFM322512ALMAR47MTAA:1
- Coincidencia:76 [Mate]: hw_DAA - PCB Power:1 ↔ TFM322512ALMAR47MTAA:2
- Coincidencia:77 [Mate]: hw_DAA - PCB Power:1 ↔ TFM322512ALMAR22MTAA:3
- Coincidencia:78 [Mate]: hw_DAA - PCB Power:1 ↔ TPS54116QRTWTQ1:1
- Coincidencia:79 [Mate]: hw_DAA - PCB Power:1 ↔ TPS62873QWRXSRQ1:1
- Coincidencia:80 [Mate]: hw_DAA - PCB Power:1 ↔ TS5A23157TDGSRQ1:1
- Coincidencia:81 [Mate]: hw_DAA - PCB Power:1 ↔ TS5A23157TDGSRQ1:1
- Coincidencia:82 [Mate]: hw_DAA - PCB Power:1 ↔ EMK212BBJ106KGHT:4
- Coincidencia:83 [Mate]: hw_DAA - PCB Power:1 ↔ EMK212BBJ106KGHT:3
- Coincidencia:84 [Mate]: hw_DAA - PCB Power:1 ↔ EMK212BBJ106KGHT:1
- Coincidencia:85 [Mate]: hw_DAA - PCB Power:1 ↔ EMK212BBJ106KGHT:2
- Coincidencia:86 [Mate]: hw_DAA - PCB Power:1 ↔ GCM32EC71A476KE02K:8
- Coincidencia:87 [Mate]: hw_DAA - PCB Power:1 ↔ GCM32EC71A476KE02K:9
- Coincidencia:88 [Mate]: hw_DAA - PCB Power:1 ↔ GCM32EC71A476KE02K:10
- Coincidencia:89 [Mate]: hw_DAA - PCB Power:1 ↔ GRT32ER60J107ME13L:1
- Ángulo:1 [Angle] (0 deg): hw_DAA - PCB Power:1 ↔ GRT32ER60J107ME13L:1
- Ángulo:2 [Angle] (0 deg): hw_DAA - PCB Power:1 ↔ GCM32EC71A476KE02K:10
- Coincidencia:90 [Mate]: hw_DAA - PCB Power:1 ↔ GRT32ER60J107ME13L:2
- Ángulo:3 [Angle] (0 deg): hw_DAA - PCB Power:1 ↔ GRT32ER60J107ME13L:2
- Coincidencia:91 [Mate]: hw_DAA - PCB Power:1 ↔ CGA6P3X7S1H685M250AB:1
- Coincidencia:92 [Mate]: hw_DAA - PCB Power:1 ↔ CGA6P3X7S1H685M250AB:2
- Coincidencia:93 [Mate]: hw_DAA - PCB Power:1 ↔ GCM32EC71A476KE02K:11
- Coincidencia:94 [Mate]: hw_DAA - PCB Power:1 ↔ GCM32EC71A476KE02K:12
- Coincidencia:95 [Mate]: hw_DAA - PCB Power:1 ↔ GCM32EC71A476KE02K:13
- Coincidencia:96 [Mate]: hw_DAA - PCB Power:1 ↔ GRM31CC72A475ME11L:1
- Coincidencia:97 [Mate]: hw_DAA - PCB Power:1 ↔ GRM31CC72A475ME11L:2
- Ángulo:4 [Angle] (0 deg): hw_DAA - PCB Power:1 ↔ GRM31CC72A475ME11L:2
- Ángulo:5 [Angle] (0 deg): hw_DAA - PCB Power:1 ↔ GRM31CC72A475ME11L:1
- Coincidencia:98 [Mate]: hw_DAA - PCB Power:1 ↔ GRT32ER60J107ME13L:3
- Ángulo:6 [Angle] (0 deg): hw_DAA - PCB Power:1 ↔ GRT32ER60J107ME13L:3
- Coincidencia:99 [Mate]: hw_DAA - PCB Power:1 ↔ GCM32EC71A476KE02K:14
- Ángulo:7 [Angle] (0 deg): hw_DAA - PCB Power:1 ↔ GCM32EC71A476KE02K:14
- Coincidencia:100 [Mate]: hw_DAA - PCB Power:1 ↔ GRM31CC72A475ME11L:4
- Coincidencia:101 [Mate]: hw_DAA - PCB Power:1 ↔ GRM31CC72A475ME11L:3
- Ángulo:8 [Angle] (0 deg): hw_DAA - PCB Power:1 ↔ GRM31CC72A475ME11L:3
- Ángulo:9 [Angle] (0 deg): hw_DAA - PCB Power:1 ↔ GRM31CC72A475ME11L:4
- Coincidencia:102 [Mate]: hw_DAA - PCB Power:1 ↔ TPS57112CQRTERQ1:1
- Coincidencia:103 [Mate]: hw_DAA - PCB Power:1 ↔ TPS57112CQRTERQ1:2
- Coincidencia:104 [Mate]: hw_DAA - PCB Power:1 ↔ TPS74525PQWDRBRQ1:1
- Coincidencia:105 [Mate]: hw_DAA - PCB Power:1 ↔ ECS-.327-12.5-34QCS-TR:1
- Coincidencia:106 [Mate]: hw_DAA - PCB Power:1 ↔ RCLAMP3324PQTCT:2
- Coincidencia:107 [Mate]: hw_DAA - PCB Power:1 ↔ RCLAMP3324PQTCT:1
- Ángulo:10 [Angle] (0 deg): hw_DAA - PCB Power:1 ↔ RCLAMP3324PQTCT:1
- Ángulo:11 [Angle] (0 deg): hw_DAA - PCB Power:1 ↔ RCLAMP3324PQTCT:2
- Coincidencia:108 [Mate]: hw_DAA - PCB Power:1 ↔ CRCW12061R00FKEAHP:1
- Coincidencia:109 [Mate]: hw_DAA - PCB Power:1 ↔ CRCW12061R00FKEAHP:2
- Ángulo:12 [Angle] (0 deg): hw_DAA - PCB Power:1 ↔ CRCW12061R00FKEAHP:2
- Ángulo:13 [Angle] (0 deg): hw_DAA - PCB Power:1 ↔ CRCW12061R00FKEAHP:1
- Tangente:1: hw_DAA - PCB Power:1 ↔ CMB02070X1000GB200:1
- Ángulo:14 [Angle] (0 deg): hw_DAA - PCB Power:1 ↔ CMB02070X1000GB200:1
- Coincidencia:110 [Mate]: hw_DAA - PCB Power:1 ↔ CGA3E1X7S1C225K080AC:1
- Ángulo:15 [Angle] (0 deg): hw_DAA - PCB Power:1 ↔ CGA3E1X7S1C225K080AC:1
- Coincidencia:111 [Mate]: hw_DAA - PCB Power:1 ↔ CGA3E1X7S1C225K080AC:2
- Coincidencia:112 [Mate]: hw_DAA - PCB Power:1 ↔ CGA3E1X7S1C225K080AC:3
- Coincidencia:113 [Mate]: hw_DAA - PCB Power:1 ↔ CGA3E1X7S1C225K080AC:4
- Coincidencia:114 [Mate]: hw_DAA - PCB Power:1 ↔ CGA3E1X7S1C225K080AC:5
- Coincidencia:115 [Mate]: hw_DAA - PCB Power:1 ↔ CGA3E1X7S1C225K080AC:6
- Coincidencia:116 [Mate]: hw_DAA - PCB Power:1 ↔ EMK212BBJ106KGHT:5
- Ángulo:16 [Angle] (0 deg): hw_DAA - PCB Power:1 ↔ EMK212BBJ106KGHT:5
- Coincidencia:117 [Mate]: hw_DAA - PCB Power:1 ↔ GCM1555C1H120JA16J:2
- Coincidencia:118 [Mate]: hw_DAA - PCB Power:1 ↔ GCM1555C1H120JA16J:1
- Coincidencia:119 [Mate]: hw_DAA - PCB Power:1 ↔ CGA2B3X7R1H104K050BD:1
- Coincidencia:120 [Mate]: hw_DAA - PCB Power:1 ↔ GRT188C81A106ME13D:1
- Coincidencia:121 [Mate]: hw_DAA - PCB Power:1 ↔ GRT188C81A106ME13D:2
- Ángulo:17 [Angle] (0 deg): hw_DAA - PCB Power:1 ↔ GRT188C81A106ME13D:2
- Coincidencia:122 [Mate]: hw_DAA - PCB Power:1 ↔ GRT188C81A106ME13D:3
- Coincidencia:123 [Mate]: hw_DAA - PCB Power:1 ↔ GRT188C81A106ME13D:4
- Coincidencia:124 [Mate]: hw_DAA - PCB Power:1 ↔ HMJ107BB7104KAHT:1
- Ángulo:18 [Angle] (0 deg): hw_DAA - PCB Power:1 ↔ HMJ107BB7104KAHT:1
- Coincidencia:125 [Mate]: hw_DAA - PCB Power:1 ↔ CAPC-0402-T0.55-BN:1
- Coincidencia:126 [Mate]: hw_DAA - PCB Power:1 ↔ CGA2B3X7R1H104K050BD:2
- Ángulo:19 [Angle] (0 deg): hw_DAA - PCB Power:1 ↔ CGA2B3X7R1H104K050BD:2
- Coincidencia:127 [Mate]: hw_DAA - PCB Power:1 ↔ HMJ107BB7104KAHT:2
- Ángulo:20 [Angle] (0 deg): hw_DAA - PCB Power:1 ↔ HMJ107BB7104KAHT:2
- Coincidencia:128 [Mate]: hw_DAA - PCB Power:1 ↔ HMJ107BB7104KAHT:3
- Coincidencia:129 [Mate]: hw_DAA - PCB Power:1 ↔ GCM1555C1H121JA16D:1
- Coincidencia:130 [Mate]: hw_DAA - PCB Power:1 ↔ CAPC-0402-T0.55-BN:2
- Coincidencia:131 [Mate]: hw_DAA - PCB Power:1 ↔ CGA2B3X7R1H104K050BD:3
- Coincidencia:132 [Mate]: hw_DAA - PCB Power:1 ↔ HMJ107BB7104KAHT:4
- Coincidencia:133 [Mate]: hw_DAA - PCB Power:1 ↔ ERJ-2GE0R00X:1
- Coincidencia:134 [Mate]: hw_DAA - PCB Power:1 ↔ ERJ-2RKF2002X:1
- Coincidencia:135 [Mate]: hw_DAA - PCB Power:1 ↔ CRCW04028K66FKTD:1
- Coincidencia:136 [Mate]: hw_DAA - PCB Power:1 ↔ ERJ-2RKF1543X:1
- Coincidencia:137 [Mate]: hw_DAA - PCB Power:1 ↔ RESC-0402:1
- Coincidencia:138 [Mate]: hw_DAA - PCB Power:1 ↔ RESC-0402:2
- Coincidencia:139 [Mate]: hw_DAA - PCB Power:1 ↔ ERJ-2RKF1002X:1
- Ángulo:21 [Angle] (0 deg): hw_DAA - PCB Power:1 ↔ ERJ-2RKF1002X:1
- Coincidencia:140 [Mate]: hw_DAA - PCB Power:1 ↔ ERJ-2RKF1002X:2
- Ángulo:22 [Angle] (0 deg): hw_DAA - PCB Power:1 ↔ ERJ-2RKF1002X:2
- Coincidencia:141 [Mate]: hw_DAA - PCB Power:1 ↔ CLP-105-02-F-D-BE:1
- Ángulo:23 [Angle] (0 deg): hw_DAA - PCB Power:1 ↔ CLP-105-02-F-D-BE:1
- Coincidencia:149 [Mate]: hw_DAA - PCB Power:1 ↔ GRT31CC81C226KE01L:1
- Ángulo:24 [Angle] (0 deg): hw_DAA - PCB Power:1 ↔ GRT31CC81C226KE01L:1
- [Mate]: hw_DAA - PCB Power:1 ↔ WP-SMRA Redcube (M2) 746630200:2
- Coincidencia:151 [Mate]: hw_DAA - PCB Power:1 ↔ WP-SMRA Redcube (M2) 7466302:2
- [Mate]: hw_DAA - PCB Power:1 ↔ WP-SMRA Redcube (M2) 746630200:3
- Ángulo:25 [Angle] (0 deg): hw_DAA - PCB Power:1 ↔ WP-SMRA Redcube (M2) 7466302:2
- Coincidencia:153 [Mate]: hw_DAA - PCB Power:1 ↔ WP-SMRA Redcube (M2) 746630200:1
- Ángulo:26 [Angle] (0 deg): hw_DAA - PCB Power:1 ↔ WP-SMRA Redcube (M2) 746630200:1
- Coincidencia:154 [Mate]: hw_DAA - PCB Power:1 ↔ LM5146QRGYRQ1:1
- Coincidencia:155 [Mate]: hw_DAA - PCB Power:1 ↔ TCA9517DGKRQ1:1
- Coincidencia:156 [Mate]: hw_DAA - PCB Power:1 ↔ TCA9517DGKRQ1:1
- Coincidencia:157 [Mate]: hw_DAA - PCB Power:1 ↔ DMN2710UTQ-7:1
- Coincidencia:158 [Mate]: hw_DAA - PCB Power:1 ↔ DMN2710UTQ-7:2
- Coincidencia:159 [Mate]: hw_DAA - PCB Power:1 ↔ DMN2710UTQ-7:4
- Coincidencia:160 [Mate]: hw_DAA - PCB Power:1 ↔ DMN2710UTQ-7:6
- Coincidencia:161 [Mate]: hw_DAA - PCB Power:1 ↔ DMN2710UTQ-7:3
- Coincidencia:162 [Mate]: hw_DAA - PCB Power:1 ↔ DMN2710UTQ-7:5
- Ángulo:27 [Angle] (0 deg): hw_DAA - PCB Power:1 ↔ DMN2710UTQ-7:3
- Ángulo:28 [Angle] (0 deg): hw_DAA - PCB Power:1 ↔ DMN2710UTQ-7:5
- Coincidencia:163 [Mate]: hw_DAA - PCB Power:1 ↔ DMN2710UTQ-7:7
- Coincidencia:164 [Mate]: hw_DAA - PCB Power:1 ↔ DMN2710UTQ-7:8
- Coincidencia:165 [Mate]: hw_DAA - PCB Power:1 ↔ BSS123NH6327XTSA1:1
- Ángulo:29 [Angle] (0 deg): hw_DAA - PCB Power:1 ↔ BSS123NH6327XTSA1:1
- Coincidencia:166 [Mate]: hw_DAA - PCB Power:1 ↔ BZD27C10P-HE3-08:1
- Ángulo:30 [Angle] (0 deg): hw_DAA - PCB Power:1 ↔ BZD27C10P-HE3-08:1
- Coincidencia:167 [Mate]: hw_DAA - PCB Power:1 ↔ BZD27C10P-HE3-08:2
- Coincidencia:168 [Mate]: hw_DAA - PCB Power:1 ↔ CGA3E1X7S1C225K080AC:7
- Ángulo:31 [Angle] (0 deg): hw_DAA - PCB Power:1 ↔ CGA3E1X7S1C225K080AC:7
- Coincidencia:169 [Mate]: hw_DAA - PCB Power:1 ↔ CGA3E1X7S1C225K080AC:8
- Coincidencia:170 [Mate]: hw_DAA - PCB Power:1 ↔ CGA3E1X7S1C225K080AC:9
- Coincidencia:171 [Mate]: hw_DAA - PCB Power:1 ↔ CGA3E1X7S1C225K080AC:10
- Coincidencia:172 [Mate]: hw_DAA - PCB Power:1 ↔ C0603C105K4RACAUTO:1
- Coincidencia:173 [Mate]: hw_DAA - PCB Power:1 ↔ CGA2B1X7S1C474K050BC:1
- Coincidencia:174 [Mate]: hw_DAA - PCB Power:1 ↔ CGA3E1X7S1C225K080AC:11
- Ángulo:32 [Angle] (0 deg): hw_DAA - PCB Power:1 ↔ CGA3E1X7S1C225K080AC:11
- Coincidencia:175 [Mate]: hw_DAA - PCB Power:1 ↔ CGA3E1X7S1C225K080AC:12
- Coincidencia:176 [Mate]: hw_DAA - PCB Power:1 ↔ CGA3E1X7S1C225K080AC:13
- Coincidencia:177 [Mate]: hw_DAA - PCB Power:1 ↔ CAPC-0402-T0.55-BN:3
- Ángulo:33 [Angle] (0 deg): hw_DAA - PCB Power:1 ↔ CAPC-0402-T0.55-BN:3
- Coincidencia:178 [Mate]: hw_DAA - PCB Power:1 ↔ GCM155R71C563KA55J:1
- Coincidencia:179 [Mate]: hw_DAA - PCB Power:1 ↔ C0402C822K4RACAUTO:1
- Coincidencia:180 [Mate]: hw_DAA - PCB Power:1 ↔ GCG155R71H821KA01D:1
- Coincidencia:181 [Mate]: hw_DAA - PCB Power:1 ↔ GCM155R71H391KA37D:1
- Ángulo:34 [Angle] (0 deg): hw_DAA - PCB Power:1 ↔ GCM155R71H391KA37D:1
- Coincidencia:182 [Mate]: hw_DAA - PCB Power:1 ↔ HMJ107BB7104KAHT:5
- Ángulo:35 [Angle] (0 deg): hw_DAA - PCB Power:1 ↔ HMJ107BB7104KAHT:5
- Coincidencia:183 [Mate]: hw_DAA - PCB Power:1 ↔ 06031A6R8J4T4A:1
- Ángulo:36 [Angle] (0 deg): hw_DAA - PCB Power:1 ↔ 06031A6R8J4T4A:1
- Coincidencia:184 [Mate]: hw_DAA - PCB Power:1 ↔ CGA3E1X7S1C225K080AC:14
- Ángulo:37 [Angle] (0 deg): hw_DAA - PCB Power:1 ↔ CGA3E1X7S1C225K080AC:14
- Coincidencia:185 [Mate]: hw_DAA - PCB Power:1 ↔ C0603X272J5GAC7867:1
- Ángulo:38 [Angle] (0 deg): hw_DAA - PCB Power:1 ↔ C0603X272J5GAC7867:1
- Coincidencia:186 [Mate]: hw_DAA - PCB Power:1 ↔ CAPC-0402-T0.55-BN:4
- Ángulo:39 [Angle] (0 deg): hw_DAA - PCB Power:1 ↔ CAPC-0402-T0.55-BN:4
- Coincidencia:187 [Mate]: hw_DAA - PCB Power:1 ↔ HMJ107BB7104KAHT:6
- Coincidencia:188 [Mate]: hw_DAA - PCB Power:1 ↔ CAPC-0402-T0.55-BN:5
- Coincidencia:189 [Mate]: hw_DAA - PCB Power:1 ↔ C0402C822K4RACAUTO:2
- Ángulo:40 [Angle] (0 deg): hw_DAA - PCB Power:1 ↔ C0402C822K4RACAUTO:2
- Coincidencia:190 [Mate]: hw_DAA - PCB Power:1 ↔ CGA2B1X7R1V224K050BC:1
- Coincidencia:191 [Mate]: hw_DAA - PCB Power:1 ↔ GRT155R71H331KE01D:1
- Coincidencia:192 [Mate]: hw_DAA - PCB Power:1 ↔ 04025A220C4T2A:1
- Coincidencia:193 [Mate]: hw_DAA - PCB Power:1 ↔ GCM155R71H332KA37J:1
- Ángulo:41 [Angle] (0 deg): hw_DAA - PCB Power:1 ↔ GCM155R71H332KA37J:1
- Ángulo:42 [Angle] (90 deg): hw_DAA - PCB Power:1 ↔ GCM155R71H332KA37J:2
- Coincidencia:195 [Mate]: hw_DAA - PCB Power:1 ↔ C0603X272J5GAC7867:2
- Ángulo:43 [Angle] (0 deg): hw_DAA - PCB Power:1 ↔ C0603X272J5GAC7867:2
- Coincidencia:196 [Mate]: hw_DAA - PCB Power:1 ↔ GCQ1555C1H100FB01D:1
- Ángulo:44 [Angle] (0 deg): hw_DAA - PCB Power:1 ↔ GCQ1555C1H100FB01D:1
- Coincidencia:197 [Mate]: hw_DAA - PCB Power:1 ↔ GCM155R72A472MA37D:1
- Coincidencia:198 [Mate]: hw_DAA - PCB Power:1 ↔ 04025A220C4T2A:2
- Coincidencia:200 [Mate]: hw_DAA - PCB Power:1 ↔ CAPC-0402-T0.55-BN:7
- Coincidencia:201 [Mate]: hw_DAA - PCB Power:1 ↔ AC0805FR-0749K9L:1
- Coincidencia:202 [Mate]: hw_DAA - PCB Power:1 ↔ AC0805FR-0749K9L:2
- Coincidencia:203 [Mate]: hw_DAA - PCB Power:1 ↔ RESC-0402:3
- Ángulo:45 [Angle] (0 deg): hw_DAA - PCB Power:1 ↔ RESC-0402:3
- Coincidencia:204 [Mate]: hw_DAA - PCB Power:1 ↔ ERJ-2RKF1003X:1
- Ángulo:46 [Angle] (0 deg): hw_DAA - PCB Power:1 ↔ ERJ-2RKF1003X:1
- Coincidencia:205 [Mate]: hw_DAA - PCB Power:1 ↔ ERJ-2RKF1003X:2
- Coincidencia:206 [Mate]: hw_DAA - PCB Power:1 ↔ ERJ-2GE0R00X:2
- Coincidencia:207 [Mate]: hw_DAA - PCB Power:1 ↔ ERJ-2GE0R00X:3
- Coincidencia:208 [Mate]: hw_DAA - PCB Power:1 ↔ ERJ-2RKF1002X:3
- Coincidencia:209 [Mate]: hw_DAA - PCB Power:1 ↔ ERJ-2RKF1002X:4
- Ángulo:47 [Angle] (0 deg): hw_DAA - PCB Power:1 ↔ ERJ-2RKF1002X:4
- Coincidencia:210 [Mate]: hw_DAA - PCB Power:1 ↔ ERJ-2GE0R00X:4
- Coincidencia:211 [Mate]: hw_DAA - PCB Power:1 ↔ ERJ-2RKF1002X:5
- Coincidencia:212 [Mate]: hw_DAA - PCB Power:1 ↔ ERJ-2GE0R00X:5
- Coincidencia:213 [Mate]: hw_DAA - PCB Power:1 ↔ ERJ-2GE0R00X:6
- Coincidencia:214 [Mate]: hw_DAA - PCB Power:1 ↔ ERJ-2GE0R00X:7
- Coincidencia:215 [Mate]: hw_DAA - PCB Power:1 ↔ ERJ-2GE0R00X:8
- Coincidencia:216 [Mate]: hw_DAA - PCB Power:1 ↔ ERJ-2GE0R00X:9
- Ángulo:48 [Angle] (0 deg): hw_DAA - PCB Power:1 ↔ ERJ-2GE0R00X:9
- Ángulo:49 [Angle] (0 deg): hw_DAA - PCB Power:1 ↔ ERJ-2GE0R00X:8
- Coincidencia:217 [Mate]: hw_DAA - PCB Power:1 ↔ ERJ-2RKF1002X:6
- Coincidencia:218 [Mate]: hw_DAA - PCB Power:1 ↔ ERJ-2RKF1002X:7
- Ángulo:50 [Angle] (0 deg): hw_DAA - PCB Power:1 ↔ ERJ-2RKF1002X:7
- Coincidencia:219 [Mate]: hw_DAA - PCB Power:1 ↔ ERJ-2RKF1002X:8
- Coincidencia:220 [Mate]: hw_DAA - PCB Power:1 ↔ ERJ-U02F4701X:1
- Coincidencia:221 [Mate]: hw_DAA - PCB Power:1 ↔ ERJ-U02F4701X:3
- Coincidencia:222 [Mate]: hw_DAA - PCB Power:1 ↔ ERJ-U02F4701X:2
- Coincidencia:223 [Mate]: hw_DAA - PCB Power:1 ↔ ERJ-U02F4701X:4
- Ángulo:51 [Angle] (0 deg): hw_DAA - PCB Power:1 ↔ ERJ-U02F4701X:2
- Ángulo:52 [Angle] (0 deg): hw_DAA - PCB Power:1 ↔ ERJ-U02F4701X:4
- Coincidencia:224 [Mate]: hw_DAA - PCB Power:1 ↔ C0603C105K4RACAUTO:2
- Ángulo:53 [Angle] (0 deg): hw_DAA - PCB Power:1 ↔ C0603C105K4RACAUTO:2
- Coincidencia:225 [Mate]: hw_DAA - PCB Power:1 ↔ CRCW040233K0FKED:1
- Ángulo:54 [Angle] (0 deg): hw_DAA - PCB Power:1 ↔ CRCW040233K0FKED:1
- Coincidencia:226 [Mate]: hw_DAA - PCB Power:1 ↔ ERJ-2RKF1003X:3
- Coincidencia:227 [Mate]: hw_DAA - PCB Power:1 ↔ ERJ-2RKF1002X:9
- Coincidencia:228 [Mate]: hw_DAA - PCB Power:1 ↔ CRCW04028K66FKTD:2
- Coincidencia:229 [Mate]: hw_DAA - PCB Power:1 ↔ ERJ-2RKF1002X:10
- Coincidencia:230 [Mate]: hw_DAA - PCB Power:1 ↔ GSOT05C-HE3-08:1
- Coincidencia:231 [Mate]: hw_DAA - PCB Power:1 ↔ GSOT05C-HE3-08:1
- Coincidencia:232 [Mate]: hw_DAA - PCB Power:1 ↔ CGA2B3X7R1H104K050BD:4
- Coincidencia:233 [Mate]: hw_DAA - PCB Power:1 ↔ CGA2B3X7R1H104K050BD:5
- Coincidencia:234 [Mate]: hw_DAA - PCB Power:1 ↔ ERJ-2RKF1002X:12
- Coincidencia:235 [Mate]: hw_DAA - PCB Power:1 ↔ RESC-0402:4
- Coincidencia:236 [Mate]: hw_DAA - PCB Power:1 ↔ ERJ-2RKF1002X:11
- Coincidencia:237 [Mate]: hw_DAA - PCB Power:1 ↔ ERJ-U02F4701X:6
- Coincidencia:238 [Mate]: hw_DAA - PCB Power:1 ↔ ERJ-U02F4701X:5
- Coincidencia:239 [Mate]: hw_DAA - PCB Power:1 ↔ ERJ-U02F4701X:7
- Coincidencia:240 [Mate]: hw_DAA - PCB Power:1 ↔ ERJ-U02F4701X:8
- Coincidencia:241 [Mate]: hw_DAA - PCB Power:1 ↔ ERJ-2RKF9090X:1
- Coincidencia:242 [Mate]: hw_DAA - PCB Power:1 ↔ CRCW060315K0FKEA:1
- Coincidencia:243 [Mate]: hw_DAA - PCB Power:1 ↔ CRCW06036K19FKEA:1
- Coincidencia:244 [Mate]: hw_DAA - PCB Power:1 ↔ CRCW06036K19FKEA:2
- Coincidencia:245 [Mate]: hw_DAA - PCB Power:1 ↔ ERJ-2RKF1002X:13
- Coincidencia:250 [Mate]: hw_DAA - PCB Power:1 ↔ RESC-0402:5
- Coincidencia:251 [Mate]: hw_DAA - PCB Power:1 ↔ ERJ-2RKF1003X:5
- Coincidencia:252 [Mate]: hw_DAA - PCB Power:1 ↔ ERJ-2RKF1003X:6
- Coincidencia:253 [Mate]: hw_DAA - PCB Power:1 ↔ AC0402FR-0797K6L:1
- Coincidencia:254 [Mate]: hw_DAA - PCB Power:1 ↔ CRCW040278K7FKTD:1
- Coincidencia:255 [Mate]: hw_DAA - PCB Power:1 ↔ RESC-0402:6
- Coincidencia:256 [Mate]: hw_DAA - PCB Power:1 ↔ CRCW04023K40FKED:1
- Coincidencia:257 [Mate]: hw_DAA - PCB Power:1 ↔ CRCW0402133RFKED:1
- Coincidencia:258 [Mate]: hw_DAA - PCB Power:1 ↔ RK73H1ETTP1802F:1
- Coincidencia:259 [Mate]: hw_DAA - PCB Power:1 ↔ ERJ-2RKF1002X:14
- Coincidencia:260 [Mate]: hw_DAA - PCB Power:1 ↔ ERJ-2RKF1501X:1
- Ángulo:55 [Angle] (0 deg): hw_DAA - PCB Power:1 ↔ ERJ-2RKF1501X:1
- Coincidencia:261 [Mate]: hw_DAA - PCB Power:1 ↔ CRCW040239K2FKED:1
- Coincidencia:262 [Mate]: hw_DAA - PCB Power:1 ↔ ERJ-2RKF1003X:8
- Ángulo:56 [Angle] (0 deg): hw_DAA - PCB Power:1 ↔ ERJ-2RKF1003X:8
- Coincidencia:263 [Mate]: hw_DAA - PCB Power:1 ↔ CRCW06032R10FKEA:1
- Coincidencia:264 [Mate]: hw_DAA - PCB Power:1 ↔ CRCW0603931RFKEA:1
- Ángulo:57 [Angle] (0 deg): hw_DAA - PCB Power:1 ↔ CRCW0603931RFKEA:1
- Nivelación:1 [Flush]: hw_DAA - PCB Power:1 ↔ WP-SMRA Redcube (M2) 7466302:2
- [Flush] (1.742 mm): hw_DAA - PCB Power:1 ↔ WP-SMRA Redcube (M2) 746630200:2
- [Flush] (1.742 mm): hw_DAA - PCB Power:1 ↔ WP-SMRA Redcube (M2) 746630200:3
- Nivelación:4 [Flush] (24.692 mm): hw_DAA - PCB Power:1 ↔ WP-SMRA Redcube (M2) 746630200:1
- Ángulo:58 [Angle] (0 deg): hw_DAA - PCB Power:1 ↔ GCM32EC71A476KE02K:5
- Ángulo:59 [Angle] (0 deg): hw_DAA - PCB Power:1 ↔ GCM32EC71A476KE02K:6
- Ángulo:60 [Angle] (0 deg): hw_DAA - PCB Power:1 ↔ GCM32EC71A476KE02K:7
- Ángulo:61 [Angle] (0 deg): hw_DAA - PCB Power:1 ↔ GCM32EC71A476KE02K:19
- Ángulo:62 [Angle] (0 deg): hw_DAA - PCB Power:1 ↔ GCM32EC71A476KE02K:20
- Ángulo:63 [Angle] (0 deg): hw_DAA - PCB Power:1 ↔ GCM32EC71A476KE02K:15
- Coincidencia:266 [Mate]: hw_DAA - PCB Power:1 ↔ GCM32EC71A476KE02K:20
- Coincidencia:267 [Mate]: hw_DAA - PCB Power:1 ↔ GCM32EC71A476KE02K:19
- Coincidencia:268 [Mate]: hw_DAA - PCB Power:1 ↔ GCM32EC71A476KE02K:15
- Coincidencia:269 [Mate]: hw_DAA - PCB Power:1 ↔ GCM32EC71A476KE02K:18
- Coincidencia:270 [Mate]: hw_DAA - PCB Power:1 ↔ GCM32EC71A476KE02K:17
- Coincidencia:271 [Mate]: hw_DAA - PCB Power:1 ↔ GCM32EC71A476KE02K:16
- Coincidencia:272 [Mate]: hw_DAA - PCB Power:1 ↔ GCM32EC71A476KE02K:21
- Ángulo:64 [Angle] (0 deg): hw_DAA - PCB Power:1 ↔ GCM32EC71A476KE02K:16
- Ángulo:65 [Angle] (0 deg): hw_DAA - PCB Power:1 ↔ GCM32EC71A476KE02K:21
- Coincidencia:273 [Mate]: hw_DAA - PCB Power:1 ↔ GRT32ER60J107ME13L:4
- Coincidencia:274 [Mate]: hw_DAA - PCB Power:1 ↔ CGA2B3X7R1H104K050BD:6
- Coincidencia:275 [Mate]: hw_DAA - PCB Power:1 ↔ C0603X272J5GAC7867:3
- Coincidencia:276 [Mate]: hw_DAA - PCB Power:1 ↔ ERJ-2RKF1003X:4
- Ángulo:66 [Angle] (0 deg): hw_DAA - PCB Power:1 ↔ ERJ-2RKF1003X:4
- Coincidencia:277 [Mate]: hw_DAA - PCB Power:1 ↔ CRGP0402F47K:1
- Coincidencia:278 [Mate]: hw_DAA - PCB Power:1 ↔ CAPC-0402-T0.55-BN:6
- Ángulo:67 [Angle] (0 deg): hw_DAA - PCB Power:1 ↔ CAPC-0402-T0.55-BN:6
- Coincidencia:279 [Mate]: hw_DAA - PCB Power:1 ↔ CGA2B3X7R1H104K050BD:7
- [Mate] (-35.192 mm): hw_DAA - PCB Power:1 ↔ WP-SMRA Redcube (M2) 746630200:3
- Coincidencia:281 [Mate] (-12.01 mm): hw_DAA - PCB Power:1 ↔ WP-SMRA Redcube (M2) 7466302:2
- [Mate] (-45.1 mm): hw_DAA - PCB Power:1 ↔ WP-SMRA Redcube (M2) 746630200:2
- Coincidencia:283 [Mate] (-7.517 mm): hw_DAA - PCB Power:1 ↔ WP-SMRA Redcube (M2) 746630200:1
- Coincidencia:284 [Mate]: hw_DAA - PCB Power:1 ↔ ERJ-2RKF1003X:9
- Ángulo:68 [Angle] (0 deg): hw_DAA - PCB Power:1 ↔ ERJ-2RKF1003X:9
- Coincidencia:285 [Mate]: hw_DAA - PCB Power:1 ↔ ERJ-2RKF1003X:7
- Coincidencia:286 [Mate]: hw_DAA - PCB Power:1 ↔ GCM155R71H332KA37J:2
- Coincidencia:287 [Mate]: hw_DAA - PCB Power:1 ↔ CRCW0402110KFKTD:1
- Ángulo:69 [Angle] (0 deg): hw_DAA - PCB Power:1 ↔ CRCW0402110KFKTD:1
- Ángulo:70 [Angle] (0 deg): hw_DAA - PCB Power:1 ↔ ERJ-2RKF1003X:7
